# Autodesk Inventor assembly: 20-028
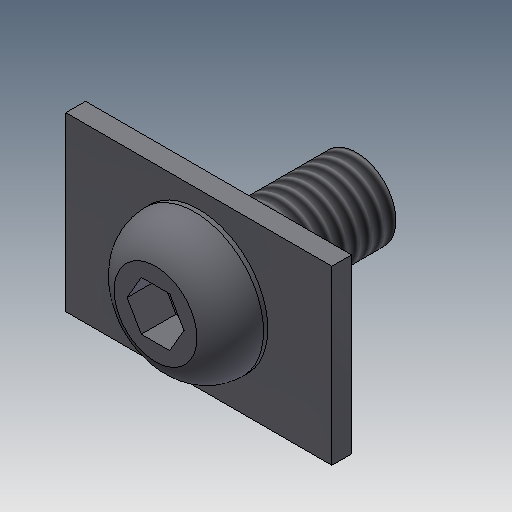
[picture p0: Inventor's stored thumbnail of the model, 512x512]
Saved by Autodesk Inventor 2018.3 (Build 223284000, 284)
## iProperties
Created: 2004-10-14
Part Number: 20-028
Document SubType Name: Assembly
Designer: Autodesk, Inc.
Manufacturer: Standard
Standards Organization: Custom
Description: FLAT PLATE FASTENING SET
Catalog Web Link: http://www.parker.com/ead/cm1.asp?cmid=809
Vendor: PARKER IPS
Mass: 16.7148 g
Surface Area: 19.5999 cm^2
Volume: 2.13199 cm^3
Density: 7.84 g/cm^3
CAGE: 1LJX3
Dept. ID: Product Design
Description #2: ---
Finish #1: ---
Finish #2: ---
Material ID: ---
Project Number: ---
Author: Autodesk, Inc.
## Documents named in this file (4)
- C:\AVAInvAPI\Workspace\Test Station\Components\20-028.iam
- C:\AVAInvAPI\Workspace\Test Station\Components\20-028Z1.ipt
- C:\AVAInvAPI\Workspace\Test Station\Components\24-116-8.ipt
- C:\workfolder\Extra Samples\Models\Test Station\Library\Parker - IPS\Fastners\2X-YYY-ZZ IPS Screws.ipt
## Components (2 placed, 2 different names)
1. 20-028Z1:1 — Insert:1
2. 24-116-8:1 — Insert:1
## Relationships (1: Insert 1)
- Insert:1: 20-028Z1:1 ↔ 24-116-8:1
